# Autodesk Inventor assembly: Motor Assembly
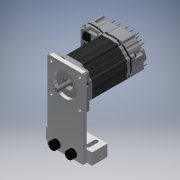
[picture p0: Inventor's stored thumbnail of the model, 180x180]
Saved by Autodesk Inventor 2016 (Build 200138000, 138)
## iProperties
Created: 2015-07-08
Part Number: Motor Assembly
Document SubType Name: Assembly
Designer: Dennis
Author: Dennis
## Documents named in this file (5)
- C:\Users\Matthew Cheung\Dropbox\Work\National Instruments\Shared Folder\NI Ball Bearing Slider Crank\CAD\Assemblies\Motor Assembly.iam
- C:\Users\Matthew Cheung\Dropbox\Work\National Instruments\Shared Folder\NI Ball Bearing Slider Crank\CAD\Motor - CPM-_ _ _ _ - 2321_-Q_.ipt
- C:\Users\Matthew Cheung\Dropbox\Work\National Instruments\Shared Folder\NI Ball Bearing Slider Crank\CAD\Motor Base.ipt
- C:\Users\Matthew Cheung\Dropbox\Work\National Instruments\Shared Folder\NI Ball Bearing Slider Crank\CAD\Motor Support.ipt
- C:\Users\Matthew Cheung\Dropbox\Work\National Instruments\Shared Folder\NI Ball Bearing Slider Crank\CAD\McMaster Parts\M5x1.25x30.ipt
## Components (5 placed, 4 different names)
1. Motor Base:1 — Mate:1, Mate:2, Mate:3
2. Motor Support:1 — Mate:1, Mate:2, Mate:3, Mate:4, Mate:5, Mate:6, Mate:7, Mate:8, Mate:9
3. Motor - CPM-_ _ _ _ - 2321_-Q_:1 — Mate:4, Mate:5
4. M5x1.25x30:1 — Mate:6, Mate:8
5. M5x1.25x30:2 — Mate:7, Mate:9
## Relationships (9: Mate 9)
- Mate:1: Motor Base:1 ↔ Motor Support:1
- Mate:2: Motor Base:1 ↔ Motor Support:1
- Mate:3: Motor Base:1 ↔ Motor Support:1
- Mate:4: Motor Support:1 ↔ Motor - CPM-_ _ _ _ - 2321_-Q_:1
- Mate:5: Motor Support:1 ↔ Motor - CPM-_ _ _ _ - 2321_-Q_:1
- Mate:6: Motor Support:1 ↔ M5x1.25x30:1
- Mate:7: Motor Support:1 ↔ M5x1.25x30:2
- Mate:8: Motor Support:1 ↔ M5x1.25x30:1
- Mate:9: Motor Support:1 ↔ M5x1.25x30:2
